# Autodesk Inventor assembly: 左前脚ユニット5
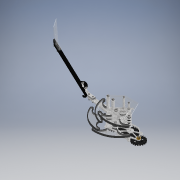
[picture p0: Inventor's stored thumbnail of the model, 180x180]
Saved by Autodesk Inventor 2020 (Build 240168000, 168)
## iProperties
Created: 2019-09-03
Part Number: 左前脚ユニット5
Document SubType Name: Assembly
Designer: 雪村
Mass: 299.669 g
Surface Area: 1628.83 cm^2
Volume: 130.463 cm^3
Density: 2.29698 g/cm^3
Author: 雪村
## Documents named in this file (30)
- C:\Users\white\Documents\SRDC\SRDC\Inventor_2017\2018年機体\2020年4年機体\左前脚ユニット5.iam
- C:\Users\white\Documents\SRDC\SRDC\Inventor_2017\2018年機体\2020年4年機体\脚内フレーム5.ipt
- C:\Users\white\Documents\SRDC\SRDC\Inventor_2017\2018年機体\2020年4年機体\脚クランク1.iam
- C:\Users\white\Documents\SRDC\SRDC\Inventor_2017\2018年機体\2020年4年機体\脚最終段カム1.ipt
- C:\Users\white\Documents\SRDC\SRDC\Inventor_2017\2018年機体\パーツ\オイレスフランジ付き12142006.ipt
- C:\Users\white\Documents\SRDC\SRDC\Inventor_2017\2018年機体\2020年4年機体\ヘッケン＋揺動節2_MIR.iam
- C:\Users\white\Documents\SRDC\SRDC\Inventor_2017\2018年機体\2020年4年機体\脚外フレーム5.ipt
- C:\Users\white\Documents\SRDC\SRDC\Inventor_2017\2018年機体\2020年4年機体\前脚ギアトレイン5.iam
- C:\Users\white\Documents\SRDC\SRDC\Inventor_2017\2018年機体\パーツ\スペーサーm3,35.ipt
- C:\Users\white\Documents\SRDC\SRDC\Inventor_2017\2018年機体\2020年4年機体\歯車m2.z24.ipt
- C:\Users\white\Documents\SRDC\SRDC\Inventor_2017\2018年機体\2020年4年機体\前脚軸抑え1.ipt
- C:\Users\white\Documents\SRDC\SRDC\Inventor_2017\2018年機体\パーツ\スペーサーm4,35.ipt
- C:\Users\white\Documents\SRDC\SRDC\Inventor_2017\2018年機体\2020年4年機体\カウンター1.1.1.ipt
- C:\Users\white\Documents\SRDC\SRDC\Inventor_2017\2018年機体\2020年4年機体\カウンター1.2.1.ipt
- C:\Users\white\Documents\SRDC\SRDC\Inventor_2017\2018年機体\2020年4年機体\カウンター1.4.1.ipt
- C:\Users\white\Documents\SRDC\SRDC\Inventor_2017\2018年機体\パーツ\ネジ皿m3,08.ipt
- C:\Users\white\Documents\SRDC\SRDC\Inventor_2017\2018年機体\パーツ\ネジ鍋m3,08.ipt
- C:\Users\white\Documents\SRDC\SRDC\Inventor_2017\2018年機体\2020年4年機体\脚最終段カム5.ipt
- C:\Users\white\Documents\SRDC\SRDC\Inventor_2017\2018年機体\パーツ\オイレスフランジ付き12142003.ipt
- C:\Users\white\Documents\SRDC\SRDC\Inventor_2017\2018年機体\パーツ\ネジ鍋m3,20.ipt
- C:\Users\white\Documents\SRDC\SRDC\Inventor_2017\2018年機体\パーツ\ネジ鍋m3,18.ipt
- C:\Users\white\Documents\SRDC\SRDC\Inventor_2017\2018年機体\パーツ\ネジ鍋m4,08.ipt
- C:\Users\white\Documents\SRDC\SRDC\Inventor_2017\2018年機体\パーツ\ネジ鍋m4,14.ipt
- C:\Users\white\Documents\SRDC\SRDC\Inventor_2017\2018年機体\パーツ\ナイロンナットm3.ipt
- C:\Users\white\Documents\SRDC\SRDC\Inventor_2017\2018年機体\alternative\カウンター3.ipt
- C:\Users\white\Documents\SRDC\SRDC\Inventor_2017\2018年機体\パーツ\スペーサーm3,6.ipt
- C:\Users\white\Documents\SRDC\SRDC\Inventor_2017\2018年機体\パーツ\スペーサーm3,10.ipt
- C:\Users\white\Documents\SRDC\SRDC\Inventor_2017\2018年機体\パーツ\ベアリングフランジ付き0610.3t.ipt
- C:\Users\white\Documents\SRDC\SRDC\Inventor_2017\2018年機体\パーツ\ワッシャー6.2,14.0.5t.ipt
- C:\Users\white\Documents\SRDC\SRDC\Inventor_2017\2018年機体\パーツ\ネジ鍋m3,16.ipt
## Components (59 placed, 29 different names)
1. 脚内フレーム5:1 — メイト:1, メイト:2, メイト:3, メイト:4, 挿入:16, 挿入:18, 挿入:19, 挿入:20, 挿入:34, 挿入:36, メイト:5, 挿入:43, 挿入:44, 挿入:48, 挿入:49, 挿入:81, 挿入:83, 挿入:84, 挿入:85
2. 脚クランク1:1 [sub-assembly] — 挿入:1, 挿入:2, 挿入:3, 挿入:5, 挿入:6, 挿入:7, 挿入:8, 挿入:88
3. 脚最終段カム1:1 — 挿入:1, 挿入:2, 挿入:23, 挿入:24
4. オイレスフランジ付き12142006:1 — 挿入:3, 挿入:16
5. ヘッケン＋揺動節2_MIR:1 [sub-assembly] — メイト:1, 挿入:5
6. ヘッケン＋揺動節2_MIR:2 [sub-assembly] — 挿入:6, メイト:4
7. ヘッケン＋揺動節2_MIR:3 [sub-assembly] — 挿入:7, メイト:2
8. ヘッケン＋揺動節2_MIR:4 [sub-assembly] — 挿入:8, メイト:3
9. スペーサーm3,35:2 — 挿入:20, 挿入:21
10. スペーサーm3,35:3 — 挿入:18
11. スペーサーm3,35:4 — 挿入:19
12. 脚外フレーム5:1 — 挿入:21, 挿入:35, 挿入:45, 挿入:46, 挿入:47, 挿入:58, 挿入:82
13. 前脚ギアトレイン5:1 [sub-assembly] — 挿入:43
14. 歯車m2.z24:1 — 挿入:23, 挿入:24, 挿入:31, 挿入:32
15. スペーサーm3,10:1 — 挿入:84
16. スペーサーm3,10:2 — 挿入:85, 挿入:86
17. スペーサーm3,10:3 — 挿入:83, 挿入:87
18. 前脚軸抑え1:1 — 挿入:86, 挿入:87, 挿入:90, 挿入:91, 挿入:92
19. 脚最終段カム5:1 — 挿入:31, 挿入:32, 挿入:33, 挿入:50, 挿入:51, 挿入:52, 挿入:53
20. オイレスフランジ付き12142003:1 — 挿入:33
21. スペーサーm4,35:1 — 挿入:34, 挿入:35
22. カウンター1.1.1:1 — 挿入:36, メイト:5, 挿入:37, 挿入:38, 挿入:57, 挿入:60, 挿入:71, 挿入:72
23. カウンター1.2.1:1 — 挿入:37, 挿入:38, 挿入:61, 挿入:62, 挿入:63, 挿入:64, 挿入:73, 挿入:74, メイト:7
24. カウンター1.4.1:1 — 挿入:65, 挿入:66, 挿入:75, 挿入:76
25. ネジ皿m3,08:1 — 挿入:44
26. ネジ鍋m3,08:1 — 挿入:49
27. ネジ鍋m3,08:2 — 挿入:48
28. ネジ鍋m3,08:3 — 挿入:45
29. ネジ鍋m3,08:4 — 挿入:46
30. ネジ鍋m3,08:5 — 挿入:47
31. ネジ鍋m3,20:1 — 挿入:50
32. ネジ鍋m3,20:2 — 挿入:51
33. ネジ鍋m3,20:3 — 挿入:52
34. ネジ鍋m3,20:4 — 挿入:53
35. ネジ鍋m4,08:1 — 挿入:58
36. ネジ鍋m4,14:1 — 挿入:57
37. ネジ鍋m4,14:2 — 挿入:60
38. ネジ鍋m3,18:7 — 挿入:61
39. ネジ鍋m3,18:8 — 挿入:63
40. ネジ鍋m3,18:9 — 挿入:62
41. ネジ鍋m3,18:10 — 挿入:65
42. ネジ鍋m3,18:11 — 挿入:66
43. ネジ鍋m3,18:12 — 挿入:64, メイト:9
44. ナイロンナットm3:1 — 挿入:77
45. ナイロンナットm3:2 — 挿入:78
46. ナイロンナットm3:3 — 挿入:79
47. ナイロンナットm3:4 — 挿入:80
48. ナイロンナットm3:5 — 挿入:71
49. ナイロンナットm3:6 — 挿入:72
50. カウンター3:1 — 挿入:75, 挿入:76, 挿入:77, 挿入:78, メイト:7, メイト:8, メイト:10
51. スペーサーm3,6:1 — 挿入:73, 挿入:80, メイト:9, メイト:10
52. スペーサーm3,6:2 — 挿入:74, 挿入:79, メイト:8
53. スペーサーm4,35:2 — 挿入:81
54. ネジ鍋m4,08:2 — 挿入:82
55. ベアリングフランジ付き0610.3t:1 — 挿入:89
56. ワッシャー6.2,14.0.5t:1 — 挿入:88, 挿入:89
57. ネジ鍋m3,16:1 — 挿入:90
58. ネジ鍋m3,16:2 — 挿入:91
59. ネジ鍋m3,16:3 — 挿入:92
## Relationships (73: Insert 64, Mate 9)
- 挿入:1 [Insert]: 脚クランク1:1 ↔ 脚最終段カム1:1
- 挿入:2 [Insert]: 脚クランク1:1 ↔ 脚最終段カム1:1
- 挿入:3 [Insert]: 脚クランク1:1 ↔ オイレスフランジ付き12142006:1
- メイト:1 [Mate]: 脚内フレーム5:1 ↔ ヘッケン＋揺動節2_MIR:1
- 挿入:5 [Insert] (0.5 mm): 脚クランク1:1 ↔ ヘッケン＋揺動節2_MIR:1
- 挿入:6 [Insert] (0.5 mm): 脚クランク1:1 ↔ ヘッケン＋揺動節2_MIR:2
- 挿入:7 [Insert] (0.5 mm): 脚クランク1:1 ↔ ヘッケン＋揺動節2_MIR:3
- 挿入:8 [Insert] (0.5 mm): 脚クランク1:1 ↔ ヘッケン＋揺動節2_MIR:4
- メイト:2 [Mate]: 脚内フレーム5:1 ↔ ヘッケン＋揺動節2_MIR:3
- メイト:3 [Mate]: 脚内フレーム5:1 ↔ ヘッケン＋揺動節2_MIR:4
- メイト:4 [Mate]: 脚内フレーム5:1 ↔ ヘッケン＋揺動節2_MIR:2
- 挿入:16 [Insert]: 脚内フレーム5:1 ↔ オイレスフランジ付き12142006:1
- 挿入:18 [Insert]: 脚内フレーム5:1 ↔ スペーサーm3,35:3
- 挿入:19 [Insert]: 脚内フレーム5:1 ↔ スペーサーm3,35:4
- 挿入:20 [Insert]: 脚内フレーム5:1 ↔ スペーサーm3,35:2
- 挿入:21 [Insert]: スペーサーm3,35:2 ↔ 脚外フレーム5:1
- 挿入:23 [Insert]: 脚最終段カム1:1 ↔ 歯車m2.z24:1
- 挿入:24 [Insert]: 脚最終段カム1:1 ↔ 歯車m2.z24:1
- 挿入:31 [Insert]: 歯車m2.z24:1 ↔ 脚最終段カム5:1
- 挿入:32 [Insert]: 歯車m2.z24:1 ↔ 脚最終段カム5:1
- 挿入:33 [Insert]: 脚最終段カム5:1 ↔ オイレスフランジ付き12142003:1
- 挿入:34 [Insert]: 脚内フレーム5:1 ↔ スペーサーm4,35:1
- 挿入:35 [Insert]: 脚外フレーム5:1 ↔ スペーサーm4,35:1
- 挿入:36 [Insert]: 脚内フレーム5:1 ↔ カウンター1.1.1:1
- メイト:5 [Mate]: 脚内フレーム5:1 ↔ カウンター1.1.1:1
- 挿入:37 [Insert]: カウンター1.1.1:1 ↔ カウンター1.2.1:1
- 挿入:38 [Insert]: カウンター1.1.1:1 ↔ カウンター1.2.1:1
- 挿入:43 [Insert]: 脚内フレーム5:1 ↔ 前脚ギアトレイン5:1
- 挿入:44 [Insert]: 脚内フレーム5:1 ↔ ネジ皿m3,08:1
- 挿入:45 [Insert]: 脚外フレーム5:1 ↔ ネジ鍋m3,08:3
- 挿入:46 [Insert]: 脚外フレーム5:1 ↔ ネジ鍋m3,08:4
- 挿入:47 [Insert]: 脚外フレーム5:1 ↔ ネジ鍋m3,08:5
- 挿入:48 [Insert]: 脚内フレーム5:1 ↔ ネジ鍋m3,08:2
- 挿入:49 [Insert]: 脚内フレーム5:1 ↔ ネジ鍋m3,08:1
- 挿入:50 [Insert]: 脚最終段カム5:1 ↔ ネジ鍋m3,20:1
- 挿入:51 [Insert]: 脚最終段カム5:1 ↔ ネジ鍋m3,20:2
- 挿入:52 [Insert]: 脚最終段カム5:1 ↔ ネジ鍋m3,20:3
- 挿入:53 [Insert]: 脚最終段カム5:1 ↔ ネジ鍋m3,20:4
- 挿入:57 [Insert]: カウンター1.1.1:1 ↔ ネジ鍋m4,14:1
- 挿入:58 [Insert]: 脚外フレーム5:1 ↔ ネジ鍋m4,08:1
- 挿入:60 [Insert]: カウンター1.1.1:1 ↔ ネジ鍋m4,14:2
- 挿入:61 [Insert]: カウンター1.2.1:1 ↔ ネジ鍋m3,18:7
- 挿入:62 [Insert]: カウンター1.2.1:1 ↔ ネジ鍋m3,18:9
- 挿入:63 [Insert]: カウンター1.2.1:1 ↔ ネジ鍋m3,18:8
- 挿入:64 [Insert]: カウンター1.2.1:1 ↔ ネジ鍋m3,18:12
- 挿入:65 [Insert]: カウンター1.4.1:1 ↔ ネジ鍋m3,18:10
- 挿入:66 [Insert]: カウンター1.4.1:1 ↔ ネジ鍋m3,18:11
- 挿入:71 [Insert]: カウンター1.1.1:1 ↔ ナイロンナットm3:5
- 挿入:72 [Insert]: カウンター1.1.1:1 ↔ ナイロンナットm3:6
- 挿入:73 [Insert]: カウンター1.2.1:1 ↔ スペーサーm3,6:1
- 挿入:74 [Insert]: カウンター1.2.1:1 ↔ スペーサーm3,6:2
- 挿入:75 [Insert]: カウンター1.4.1:1 ↔ カウンター3:1
- 挿入:76 [Insert]: カウンター1.4.1:1 ↔ カウンター3:1
- 挿入:77 [Insert]: ナイロンナットm3:1 ↔ カウンター3:1
- 挿入:78 [Insert]: ナイロンナットm3:2 ↔ カウンター3:1
- メイト:7 [Mate]: カウンター1.2.1:1 ↔ カウンター3:1
- 挿入:79 [Insert]: ナイロンナットm3:3 ↔ スペーサーm3,6:2
- 挿入:80 [Insert]: ナイロンナットm3:4 ↔ スペーサーm3,6:1
- メイト:8 [Mate]: カウンター3:1 ↔ スペーサーm3,6:2
- メイト:9 [Mate]: ネジ鍋m3,18:12 ↔ スペーサーm3,6:1
- メイト:10 [Mate]: カウンター3:1 ↔ スペーサーm3,6:1
- 挿入:81 [Insert]: 脚内フレーム5:1 ↔ スペーサーm4,35:2
- 挿入:82 [Insert]: 脚外フレーム5:1 ↔ ネジ鍋m4,08:2
- 挿入:83 [Insert]: 脚内フレーム5:1 ↔ スペーサーm3,10:3
- 挿入:84 [Insert]: 脚内フレーム5:1 ↔ スペーサーm3,10:1
- 挿入:85 [Insert]: 脚内フレーム5:1 ↔ スペーサーm3,10:2
- 挿入:86 [Insert]: スペーサーm3,10:2 ↔ 前脚軸抑え1:1
- 挿入:87 [Insert]: スペーサーm3,10:3 ↔ 前脚軸抑え1:1
- 挿入:88 [Insert]: 脚クランク1:1 ↔ ワッシャー6.2,14.0.5t:1
- 挿入:89 [Insert]: ベアリングフランジ付き0610.3t:1 ↔ ワッシャー6.2,14.0.5t:1
- 挿入:90 [Insert]: 前脚軸抑え1:1 ↔ ネジ鍋m3,16:1
- 挿入:91 [Insert]: 前脚軸抑え1:1 ↔ ネジ鍋m3,16:2
- 挿入:92 [Insert]: 前脚軸抑え1:1 ↔ ネジ鍋m3,16:3
